# Autodesk Inventor assembly: A2017_T4_01
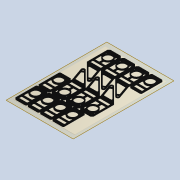
[picture p0: Inventor's stored thumbnail of the model, 180x180]
Saved by Autodesk Inventor 2022 (Build 260153000, 153)
## iProperties
Created: 2022-09-28
Part Number: A2017_T4_01
Document SubType Name: Assembly
Designer: Masato
Author: Masato
## Documents named in this file (4)
- D:\GitHub\inventor\SUSTAINA-OP\Cam\A2017_T4\A2017_T4_01.iam
- D:\GitHub\inventor\SUSTAINA-OP\Cam\DisposableBoard.ipt
- D:\GitHub\inventor\SUSTAINA-OP\UpperBody\Trunk\Trunk_neck_frame.ipt
- D:\GitHub\inventor\SUSTAINA-OP\UpperBody\Trunk\Trunk_shoulder_frame.ipt
## Components (13 placed, 3 different names)
1. DisposableBoard:1 — フラッシュ:1, フラッシュ:2, フラッシュ:3, フラッシュ:4, メイト:2, メイト:3, メイト:10
2. Trunk_neck_frame:5 — メイト:9, メイト:10, メイト:11, メイト:12
3. Trunk_shoulder_frame:6 — メイト:15, メイト:16, メイト:17, メイト:19, フラッシュ:5
4. Trunk_neck_frame:6 — メイト:18, メイト:19, フラッシュ:5
5. Trunk_neck_frame:1 — メイト:1, メイト:2, メイト:3, メイト:11
6. Trunk_neck_frame:2
7. Trunk_neck_frame:3
8. Trunk_neck_frame:4 — メイト:6
9. Trunk_shoulder_frame:1 — メイト:5, メイト:6, メイト:13, メイト:16
10. Trunk_shoulder_frame:3 — メイト:14
11. Trunk_shoulder_frame:4 — メイト:12
12. Trunk_shoulder_frame:2 — メイト:4, メイト:13, メイト:14, メイト:15
13. Trunk_shoulder_frame:5
## Component patterns: (4 elements, first: Trunk_neck_frame:1), (3 elements, first: Trunk_shoulder_frame:1), (2 elements, first: Trunk_shoulder_frame:2)
## Relationships (22: Mate 17, Flush 5)
- フラッシュ:1 [Flush]: DisposableBoard:1
- フラッシュ:2 [Flush]: DisposableBoard:1
- フラッシュ:3 [Flush]: DisposableBoard:1
- フラッシュ:4 [Flush]: DisposableBoard:1
- メイト:1 [Mate]: Trunk_neck_frame:1
- メイト:2 [Mate] (1.5 mm): DisposableBoard:1 ↔ Trunk_neck_frame:1
- メイト:3 [Mate] (1.5 mm): DisposableBoard:1 ↔ Trunk_neck_frame:1
- メイト:4 [Mate]: Trunk_shoulder_frame:2
- メイト:5 [Mate]: Trunk_shoulder_frame:1
- メイト:6 [Mate] (2.5 mm): Trunk_neck_frame:4 ↔ Trunk_shoulder_frame:1
- メイト:9 [Mate]: Trunk_neck_frame:5
- メイト:10 [Mate] (2.5 mm): DisposableBoard:1 ↔ Trunk_neck_frame:5
- メイト:11 [Mate] (2.5 mm): Trunk_neck_frame:5 ↔ Trunk_neck_frame:1
- メイト:12 [Mate] (2.5 mm): Trunk_neck_frame:5 ↔ Trunk_shoulder_frame:4
- メイト:13 [Mate] (2.5 mm): Trunk_shoulder_frame:1 ↔ Trunk_shoulder_frame:2
- メイト:14 [Mate] (2.5 mm): Trunk_shoulder_frame:3 ↔ Trunk_shoulder_frame:2
- メイト:15 [Mate] (2.5 mm): Trunk_shoulder_frame:6 ↔ Trunk_shoulder_frame:2
- メイト:16 [Mate] (2.5 mm): Trunk_shoulder_frame:6 ↔ Trunk_shoulder_frame:1
- メイト:17 [Mate]: Trunk_shoulder_frame:6
- メイト:18 [Mate]: Trunk_neck_frame:6
- メイト:19 [Mate] (2.5 mm): Trunk_shoulder_frame:6 ↔ Trunk_neck_frame:6
- フラッシュ:5 [Flush]: Trunk_shoulder_frame:6 ↔ Trunk_neck_frame:6
